# Autodesk Inventor assembly: funnel_mirrored
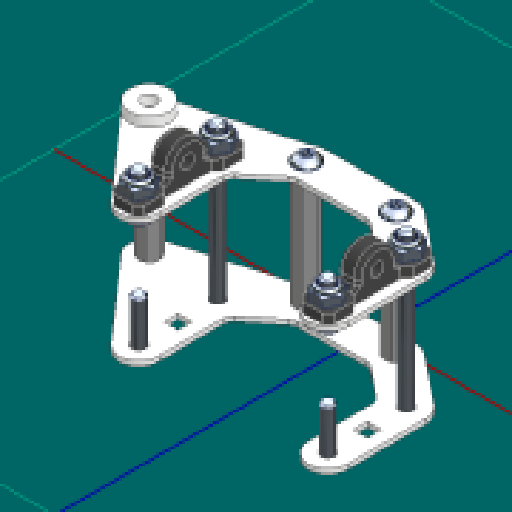
[picture p0: Inventor's stored thumbnail of the model, 512x512]
Saved by Autodesk Inventor 2025 (Build 290162000, 162)
## iProperties
Created: 2024-08-16
Part Number: funnel_mirrored
Document SubType Name: Assembly
Designer: averey
Author: averey
## Documents named in this file (14)
- C:\Users\avere\vex_robotics_high_stakes\hardware\cad\ATLAS\chassis\drive_pod\funnel_mirrored\funnel_mirrored.iam
- C:\Users\avere\vex_robotics_high_stakes\hardware\cad\ATLAS\chassis\drive_pod\funnel_mirrored\funnel_gusset_mirrored.ipt
- C:\Users\avere\vex_robotics_high_stakes\hardware\cad\VEX-CAD-Inventor\Structure\Standoff\Standoff 1.50.ipt
- C:\Users\avere\vex_robotics_high_stakes\hardware\cad\VEX-CAD-Inventor\Structure\Standoff.ipt
- C:\Users\avere\vex_robotics_high_stakes\hardware\cad\VEX-CAD-Inventor\Structure\Hardware\Screw Steel - Star\SScrew Star Smooth .290.ipt
- C:\Users\avere\vex_robotics_high_stakes\hardware\cad\VEX-CAD-Inventor\Structure\Hardware\Screw Steel - Star.ipt
- C:\Users\avere\vex_robotics_high_stakes\hardware\cad\VEX-CAD-Inventor\Structure\Hardware\Screw Shoulder Robosource\SScrew Shoulder Smooth 2.000 x .04.ipt
- C:\Users\avere\vex_robotics_high_stakes\hardware\cad\VEX-CAD-Inventor\Structure\Hardware\Screw Shoulder Robosource.ipt
- C:\Users\avere\vex_robotics_high_stakes\hardware\cad\ATLAS\chassis\drive_pod\funnel_mirrored\LS Pillow Bearing Block_mirrored.ipt
- C:\Users\avere\vex_robotics_high_stakes\hardware\cad\ATLAS\chassis\drive_pod\funnel_mirrored\Nut Thin Nylock_mirrored.ipt
- C:\Users\avere\vex_robotics_high_stakes\hardware\cad\VEX-CAD-Inventor\Structure\Hardware\Screw Shoulder Robosource\SScrew Shoulder Smooth .500 x .18.ipt
- C:\Users\avere\vex_robotics_high_stakes\hardware\cad\VEX-CAD-Inventor\Structure\Hardware\Screw Steel - Star\SScrew Star Smooth .625.ipt
- C:\Users\avere\vex_robotics_high_stakes\hardware\cad\VEX-CAD-Inventor\Motion\Spacers\Spacer Nylon .500 OD\NSpacer White .500 OD x .125.ipt
- C:\Users\avere\vex_robotics_high_stakes\hardware\cad\VEX-CAD-Inventor\Motion\Spacers\Spacer Nylon .500 OD.ipt
## Components (22 placed, 9 different names)
1. funnel_gusset_mirrored:1 — Mate:2, Mate:1, Insert:2, Insert:1, Insert:3, Insert:4, Insert:11, Insert:13, Insert:14, Insert:16, Insert:23, Insert:24
2. funnel_gusset_mirrored:2 — Mate:2, Mate:1, Insert:9, Insert:6, Insert:5, Insert:7, Insert:8, Insert:19, Insert:18
3. Standoff 1.50:1 — Insert:2
4. Standoff 1.50:2 — Insert:9, Insert:1
5. SScrew Star Smooth .290:1 — Insert:3
6. SScrew Star Smooth .290:2 — Insert:4
7. SScrew Star Smooth .290:3 — Insert:6
8. SScrew Star Smooth .290:4 — Insert:5
9. SScrew Shoulder Smooth 2.000 x .04:1 — Insert:7
10. SScrew Shoulder Smooth 2.000 x .04:2 — Insert:8
11. LS Pillow Bearing Block_mirrored:1 — Insert:11, Insert:15, Insert:21
12. Nut Thin Nylock_mirrored:1 — Insert:21
13. LS Pillow Bearing Block_mirrored:2 — Insert:13, Insert:17, Insert:22
14. Nut Thin Nylock_mirrored:2 — Insert:22
15. Nut Thin Nylock_mirrored:3 — Insert:15
16. SScrew Shoulder Smooth .500 x .18:3 — Insert:14
17. Nut Thin Nylock_mirrored:4 — Insert:17
18. SScrew Shoulder Smooth .500 x .18:4 — Insert:16
19. SScrew Star Smooth .625:5 — Insert:19
20. SScrew Star Smooth .625:6 — Insert:18
21. Standoff 1.50:3 — Insert:24
22. NSpacer White .500 OD x .125:1 — Insert:23
## Relationships (23: Insert 21, Mate 2)
- Mate:2: funnel_gusset_mirrored:1 ↔ funnel_gusset_mirrored:2
- Mate:1: funnel_gusset_mirrored:1 ↔ funnel_gusset_mirrored:2
- Insert:2: funnel_gusset_mirrored:1 ↔ Standoff 1.50:1
- Insert:9: funnel_gusset_mirrored:2 ↔ Standoff 1.50:2
- Insert:1: funnel_gusset_mirrored:1 ↔ Standoff 1.50:2
- Insert:3: funnel_gusset_mirrored:1 ↔ SScrew Star Smooth .290:1
- Insert:4: funnel_gusset_mirrored:1 ↔ SScrew Star Smooth .290:2
- Insert:6: funnel_gusset_mirrored:2 ↔ SScrew Star Smooth .290:3
- Insert:5: funnel_gusset_mirrored:2 ↔ SScrew Star Smooth .290:4
- Insert:7: funnel_gusset_mirrored:2 ↔ SScrew Shoulder Smooth 2.000 x .04:1
- Insert:8: funnel_gusset_mirrored:2 ↔ SScrew Shoulder Smooth 2.000 x .04:2
- Insert:11: funnel_gusset_mirrored:1 ↔ LS Pillow Bearing Block_mirrored:1
- Insert:13: funnel_gusset_mirrored:1 ↔ LS Pillow Bearing Block_mirrored:2
- Insert:15: LS Pillow Bearing Block_mirrored:1 ↔ Nut Thin Nylock_mirrored:3
- Insert:14 (1.5875 mm): funnel_gusset_mirrored:1 ↔ SScrew Shoulder Smooth .500 x .18:3
- Insert:17: LS Pillow Bearing Block_mirrored:2 ↔ Nut Thin Nylock_mirrored:4
- Insert:16 (1.5875 mm): funnel_gusset_mirrored:1 ↔ SScrew Shoulder Smooth .500 x .18:4
- Insert:19: funnel_gusset_mirrored:2 ↔ SScrew Star Smooth .625:5
- Insert:18: funnel_gusset_mirrored:2 ↔ SScrew Star Smooth .625:6
- Insert:21: LS Pillow Bearing Block_mirrored:1 ↔ Nut Thin Nylock_mirrored:1
- Insert:22: LS Pillow Bearing Block_mirrored:2 ↔ Nut Thin Nylock_mirrored:2
- Insert:23: funnel_gusset_mirrored:1 ↔ NSpacer White .500 OD x .125:1
- Insert:24: funnel_gusset_mirrored:1 ↔ Standoff 1.50:3
